# Autodesk Inventor assembly: A2017_T2_02
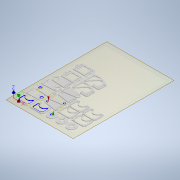
[picture p0: Inventor's stored thumbnail of the model, 180x180]
Saved by Autodesk Inventor 2020 (Build 240168000, 168)
## iProperties
Created: 2021-08-27
Part Number: A2017_T2_02
Document SubType Name: Assembly
Designer: Masato
Author: Masato
## Documents named in this file (7)
- C:\Users\L20C1118 森　圭汰\Documents\20220327_open\SUSTAINA-OP\Cam\A2017_T2_02.iam
- C:\Users\L20C1118 森　圭汰\Documents\20220327_open\SUSTAINA-OP\Cam\DisposableBoard.ipt
- C:\Users\L20C1118 森　圭汰\Documents\20220327_open\SUSTAINA-OP\LowerBody\Foot\Foot_front_frame.ipt
- C:\Users\L20C1118 森　圭汰\Documents\20220327_open\SUSTAINA-OP\LowerBody\Foot\Foot_back_frame.ipt
- C:\Users\L20C1118 森　圭汰\Documents\20220327_open\SUSTAINA-OP\LowerBody\Ankle\Ankle_back_frame.ipt
- C:\Users\L20C1118 森　圭汰\Documents\20220327_open\SUSTAINA-OP\UpperBody\Trunk\CrossRollerBearing\Inner_flange.ipt
- C:\Users\L20C1118 森　圭汰\Documents\20220327_open\SUSTAINA-OP\LowerBody\Ankle\Ankle_side_frame.ipt
## Components (20 placed, 6 different names)
1. DisposableBoard:1 — メイト:2, メイト:1, フラッシュ:1, フラッシュ:2, メイト:4, メイト:5, メイト:6, メイト:7, メイト:8, メイト:9, フラッシュ:3, フラッシュ:4, フラッシュ:5, 正接:1, 正接:2, 角度:1, 角度:2, メイト:15, メイト:20
2. Ankle_back_frame:1 — メイト:4, フラッシュ:3, フラッシュ:4, メイト:10
3. Ankle_back_frame:2 — 正接:3, メイト:12
4. Inner_flange:1 — メイト:9, 正接:2, 正接:3, 角度:2, 正接:5
5. Inner_flange:2
6. Inner_flange:3
7. Ankle_back_frame:3 — メイト:15, メイト:16, 正接:5
8. Ankle_back_frame:4
9. Ankle_back_frame:5
10. Ankle_back_frame:6
11. Foot_back_frame:2 — メイト:8, 正接:1, メイト:11, メイト:14
12. Foot_back_frame:1 — メイト:7, メイト:10, フラッシュ:5, メイト:11
13. Foot_back_frame:3 — メイト:19
14. Foot_back_frame:4
15. Foot_front_frame:1 — メイト:5, メイト:13, メイト:14, 正接:4
16. Foot_front_frame:2 — メイト:6, メイト:12, メイト:13, 角度:1, 正接:4, メイト:16
17. Foot_front_frame:3 — 正接:6
18. Foot_front_frame:4
19. Ankle_side_frame:1 — メイト:19, メイト:20, 正接:6
20. Ankle_side_frame:2
## Component patterns: (2 elements, first: Ankle_back_frame:1), (3 elements, first: Inner_flange:1), (4 elements, first: Ankle_back_frame:3), (2 elements, first: Foot_back_frame:2 + Foot_back_frame:1), (2 elements, first: Foot_front_frame:1 + Foot_front_frame:2), (2 elements, first: Ankle_side_frame:1)
## Relationships (30: Mate 17, Tangent 6, Flush 5, Angle 2)
- メイト:2 [Mate]: DisposableBoard:1
- メイト:1 [Mate]: DisposableBoard:1
- フラッシュ:1 [Flush]: DisposableBoard:1
- フラッシュ:2 [Flush]: DisposableBoard:1
- メイト:4 [Mate]: DisposableBoard:1 ↔ Ankle_back_frame:1
- メイト:5 [Mate]: DisposableBoard:1 ↔ Foot_front_frame:1
- メイト:6 [Mate]: DisposableBoard:1 ↔ Foot_front_frame:2
- メイト:7 [Mate]: DisposableBoard:1 ↔ Foot_back_frame:1
- メイト:8 [Mate]: DisposableBoard:1 ↔ Foot_back_frame:2
- メイト:9 [Mate]: DisposableBoard:1 ↔ Inner_flange:1
- フラッシュ:3 [Flush] (2 mm): DisposableBoard:1 ↔ Ankle_back_frame:1
- フラッシュ:4 [Flush] (2 mm): DisposableBoard:1 ↔ Ankle_back_frame:1
- メイト:10 [Mate] (2.5 mm): Ankle_back_frame:1 ↔ Foot_back_frame:1
- フラッシュ:5 [Flush] (2 mm): DisposableBoard:1 ↔ Foot_back_frame:1
- 正接:1 [Tangent] (2 mm): DisposableBoard:1 ↔ Foot_back_frame:2
- メイト:11 [Mate] (2.5 mm): Foot_back_frame:2 ↔ Foot_back_frame:1
- 正接:2 [Tangent] (2 mm): DisposableBoard:1 ↔ Inner_flange:1
- 正接:3 [Tangent] (2.5 mm): Ankle_back_frame:2 ↔ Inner_flange:1
- メイト:12 [Mate] (2.5 mm): Ankle_back_frame:2 ↔ Foot_front_frame:2
- メイト:13 [Mate] (2.5 mm): Foot_front_frame:1 ↔ Foot_front_frame:2
- 角度:1 [Angle] (180 deg): DisposableBoard:1 ↔ Foot_front_frame:2
- メイト:14 [Mate] (2.5 mm): Foot_back_frame:2 ↔ Foot_front_frame:1
- 正接:4 [Tangent]: Foot_front_frame:1 ↔ Foot_front_frame:2
- 角度:2 [Angle] (0 deg): DisposableBoard:1 ↔ Inner_flange:1
- メイト:15 [Mate]: DisposableBoard:1 ↔ Ankle_back_frame:3
- メイト:16 [Mate] (2.5 mm): Ankle_back_frame:3 ↔ Foot_front_frame:2
- 正接:5 [Tangent] (2.5 mm): Inner_flange:1 ↔ Ankle_back_frame:3
- メイト:19 [Mate] (2.5 mm): Foot_back_frame:3 ↔ Ankle_side_frame:1
- メイト:20 [Mate]: DisposableBoard:1 ↔ Ankle_side_frame:1
- 正接:6 [Tangent] (2.5 mm): Foot_front_frame:3 ↔ Ankle_side_frame:1
